# Autodesk Inventor assembly: motor_test
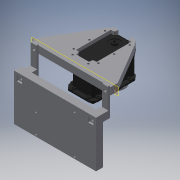
[picture p0: Inventor's stored thumbnail of the model, 180x180]
Saved by Autodesk Inventor 2018 (Build 220112000, 112)
## iProperties
Created: 2020-02-21
Part Number: motor_test
Document SubType Name: Assembly
Designer: bitbots
Author: bitbots
## Documents named in this file (5)
- C:\Users\bitbots\Desktop\bitbots_hardware\motor_tester\motor_test.iam
- C:\Users\bitbots\Desktop\bitbots_hardware\wolfgang\assembly\motors\MX106\MX-106_with_horn.iam
- C:\Users\bitbots\Desktop\bitbots_hardware\motor_tester\motor_mount.ipt
- C:\Users\bitbots\Desktop\bitbots_hardware\wolfgang\assembly\legs\foot\load_cell.ipt
- C:\Users\bitbots\Desktop\bitbots_hardware\motor_tester\base_plate.ipt
## Components (5 placed, 4 different names)
1. MX-106_with_horn:1 [sub-assembly] — Mate:5
2. motor_mount:1 — Mate:1, Mate:2, Mate:3, Mate:4, Angle:1, Angle:2, Mate:5, Flush:1, Flush:2, Flush:3
3. load_cell:1 — Mate:2, Mate:4, Angle:2
4. load_cell:2 — Mate:1, Mate:3, Angle:1, Flush:4
5. base_plate:1 — Flush:4
## Relationships (11: Mate 5, Flush 4, Angle 2)
- Mate:1: motor_mount:1 ↔ load_cell:2
- Mate:2: motor_mount:1 ↔ load_cell:1
- Mate:3: motor_mount:1 ↔ load_cell:2
- Mate:4: motor_mount:1 ↔ load_cell:1
- Angle:1 (0 deg): motor_mount:1 ↔ load_cell:2
- Angle:2 (0 deg): motor_mount:1 ↔ load_cell:1
- Mate:5: MX-106_with_horn:1 ↔ motor_mount:1
- Flush:1: motor_mount:1
- Flush:2: motor_mount:1
- Flush:3: motor_mount:1
- Flush:4: load_cell:2 ↔ base_plate:1
